# Autodesk Inventor assembly: エンコーダ取り付け
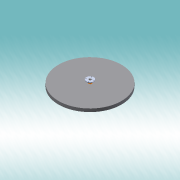
[picture p0: Inventor's stored thumbnail of the model, 180x180]
Saved by Autodesk Inventor 2015 (Build 190159000, 159)
## iProperties
Created: 2016-02-18
Part Number: エンコーダ取り付け
Document SubType Name: Assembly
Designer: buzztaka
Author: buzztaka
## Documents named in this file (10)
- C:\Users\buzztaka\Documents\tukuba\i-cart-middle_3d-model\計測輪アセンブル\新計測輪取り付け板.iam
- C:\Users\buzztaka\Documents\tukuba\i-cart-middle_3d-model\計測輪アセンブル\meh-30-pエンコーダ.ipt
- C:\Users\buzztaka\Documents\tukuba\i-cart-middle_3d-model\計測輪アセンブル\wheel-hub.ipt
- C:\Users\buzztaka\Documents\tukuba\i-cart-middle_3d-model\計測輪アセンブル\whelelcapholl.ipt
- C:\Users\buzztaka\Documents\tukuba\i-cart-middle_3d-model\計測輪アセンブル\スプリングフランジ用ワッシャー（座金）.ipt
- C:\Users\buzztaka\Documents\tukuba\i-cart-middle_3d-model\計測輪アセンブル\スプリングフランジ0.1mm.ipt
- C:\Users\buzztaka\Documents\tukuba\i-cart-middle_3d-model\計測輪アセンブル\計測輪シャフトver1.ipt
- C:\Users\buzztaka\Documents\tukuba\i-cart-middle_3d-model\計測輪アセンブル\エンコーダ取り付け板.ipt
- C:\Users\buzztaka\Documents\Inventor\Content Center Files\R2015\ja-JP\JIS B 1181 R C (2)\JIS B 1181 - M10(9).ipt
- C:\Users\buzztaka\Documents\tukuba\i-cart-middle_3d-model\計測輪アセンブル\計測輪.ipt
## Components (11 placed, 9 different names)
1. wheel-hub:1
2. whelelcapholl:1 — 挿入:18, 挿入:20
3. meh-30-pエンコーダ:1 — 挿入:11, 挿入:12, 挿入:13, 挿入:16
4. スプリングフランジ用ワッシャー（座金）:1 — 挿入:12
5. スプリングフランジ用ワッシャー（座金）:2 — 挿入:11, 挿入:14
6. スプリングフランジ用ワッシャー（座金）:3 — 挿入:13, 挿入:15
7. スプリングフランジ0.1mm:1 — 挿入:14, 挿入:15, 挿入:17
8. 計測輪シャフトver1:1 — 挿入:16, 挿入:18, 挿入:19
9. エンコーダ取り付け板:1 — 挿入:17
10. JIS B 1181 仕上程度 並 等級 2 - メートル 等級 2 仕上程度 並 M10:1 — 挿入:19
11. 計測輪:1 — 挿入:20
## Relationships (10: Insert 10)
- 挿入:11 [Insert]: meh-30-pエンコーダ:1 ↔ スプリングフランジ用ワッシャー（座金）:2
- 挿入:12 [Insert]: meh-30-pエンコーダ:1 ↔ スプリングフランジ用ワッシャー（座金）:1
- 挿入:13 [Insert]: meh-30-pエンコーダ:1 ↔ スプリングフランジ用ワッシャー（座金）:3
- 挿入:14 [Insert]: スプリングフランジ用ワッシャー（座金）:2 ↔ スプリングフランジ0.1mm:1
- 挿入:15 [Insert]: スプリングフランジ用ワッシャー（座金）:3 ↔ スプリングフランジ0.1mm:1
- 挿入:16 [Insert] (-10 mm): meh-30-pエンコーダ:1 ↔ 計測輪シャフトver1:1
- 挿入:17 [Insert]: スプリングフランジ0.1mm:1 ↔ エンコーダ取り付け板:1
- 挿入:18 [Insert]: whelelcapholl:1 ↔ 計測輪シャフトver1:1
- 挿入:19 [Insert] (2 mm): 計測輪シャフトver1:1 ↔ JIS B 1181 仕上程度 並 等級 2 - メートル 等級 2 仕上程度 並 M10:1
- 挿入:20 [Insert] (-30 mm): whelelcapholl:1 ↔ 計測輪:1
